# Autodesk Inventor assembly: Righter
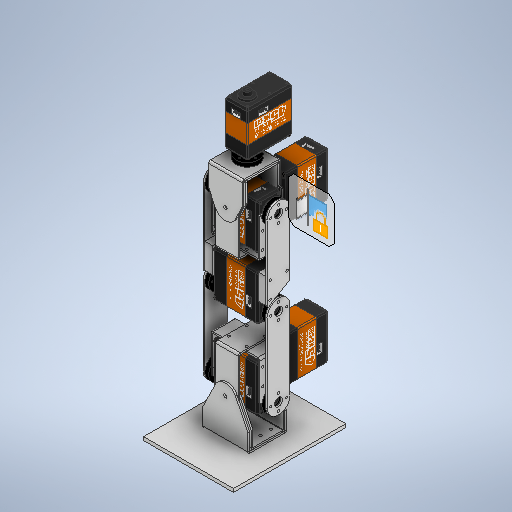
[picture p0: Inventor's stored thumbnail of the model, 512x512]
Saved by Autodesk Inventor 2025.2 (Build 292293000, 293)
## iProperties
Created: 2025-07-23
Part Number: Righter
Document SubType Name: Assembly
Designer: User
Author: User
## Documents named in this file (19)
- C:\Users\User\Documents\The Maverick's Files\College 3-3\로보인 프로젝트\RHp_Humanoid_ver1\Assembly\4_right_leg_true_final.iam
- C:\Users\User\Documents\The Maverick's Files\College 3-3\로보인 프로젝트\RHp_Humanoid_ver1\Part\HTD-45H, Horn\HTD-45H\HTD-45H.iam
- C:\Users\User\Documents\The Maverick's Files\College 3-3\로보인 프로젝트\RHp_Humanoid_ver1\Part\HTD-45H, Horn\Horn\Bottom Horn.ipt
- C:\Users\User\Documents\The Maverick's Files\College 3-3\로보인 프로젝트\RHp_Humanoid_ver1\Part\HTD-45H, Horn\Horn\Top Horn.ipt
- C:\Users\User\Documents\The Maverick's Files\College 3-3\로보인 프로젝트\RHp_Humanoid_ver1\Part\Frame\Leg\Right Leg\axis_7_top_frame.ipt
- C:\Users\User\Documents\The Maverick's Files\College 3-3\로보인 프로젝트\RHp_Humanoid_ver1\Part\Frame\Leg\Right Leg\axis_9_bottom_frame.ipt
- C:\Users\User\Documents\The Maverick's Files\College 3-3\로보인 프로젝트\RHp_Humanoid_ver1\Part\Frame\Leg\Right Leg\axis_7_supplement_frame.ipt
- C:\Users\User\Documents\The Maverick's Files\College 3-3\로보인 프로젝트\RHp_Humanoid_ver1\Part\Frame\Leg\Right Leg\axis_8_bottom_frame.ipt
- C:\Users\User\Documents\The Maverick's Files\College 3-3\로보인 프로젝트\RHp_Humanoid_ver1\Part\Frame\Leg\Right Leg\axis_8_10_connector_frame_non_powered.ipt
- C:\Users\User\Documents\The Maverick's Files\College 3-3\로보인 프로젝트\RHp_Humanoid_ver1\Part\Frame\Leg\Right Leg\axis_8_10_connector_frame_powered.ipt
- C:\Users\User\Documents\The Maverick's Files\College 3-3\로보인 프로젝트\RHp_Humanoid_ver1\Part\Frame\Leg\3D_printed_part_non_powered.ipt
- C:\Users\User\Documents\The Maverick's Files\College 3-3\로보인 프로젝트\RHp_Humanoid_ver1\Part\Frame\Leg\3D_printed_part_powered.ipt
- C:\Users\User\Documents\The Maverick's Files\College 3-3\로보인 프로젝트\RHp_Humanoid_ver1\Part\Frame\Leg\Right Leg\axis_10_11-connector_frame_non_powered.ipt
- C:\Users\User\Documents\The Maverick's Files\College 3-3\로보인 프로젝트\RHp_Humanoid_ver1\Part\Frame\Leg\Right Leg\axis_10_11-connector_frame_powered.ipt
- C:\Users\User\Documents\The Maverick's Files\College 3-3\로보인 프로젝트\RHp_Humanoid_ver1\Part\Frame\Leg\Right Leg\axis_11_top_frame.ipt
- C:\Users\User\Documents\The Maverick's Files\College 3-3\로보인 프로젝트\RHp_Humanoid_ver1\Part\Frame\Leg\Right Leg\axis_12_top_frame.ipt
- C:\Users\User\Documents\The Maverick's Files\College 3-3\로보인 프로젝트\RHp_Humanoid_ver1\Part\Frame\Leg\Right Leg\axis_12_bottom_frame(top).ipt
- C:\Users\User\Documents\The Maverick's Files\College 3-3\로보인 프로젝트\RHp_Humanoid_ver1\Part\Frame\Leg\Right Leg\axis_12_supplement_frame.ipt
- C:\Users\User\Documents\The Maverick's Files\College 3-3\로보인 프로젝트\RHp_Humanoid_ver1\Part\Frame\Leg\Right Leg\axis_12_bottom_frame(bottom).ipt
## Components (30 placed, 18 different names)
1. HTD-45H:1 [sub-assembly] — Rotational:10
2. HTD-45H:2 [sub-assembly] — Rotational:2, Rigid:5
3. HTD-45H:3 [sub-assembly] — Rigid:6, Rotational:3, Rotational:4
4. HTD-45H:4 [sub-assembly] — Rotational:5, Rotational:6, Rigid:26, Rigid:27
5. HTD-45H:5 [sub-assembly] — Rigid:16, Rotational:7, Rotational:8
6. HTD-45H:6 [sub-assembly] — Rotational:9, Rigid:19
7. Bottom Horn:3 — Rotational:3, Rigid:24
8. Bottom Horn:4 — Rotational:5, Rigid:15
9. Bottom Horn:5 — Rotational:8, Rigid:18
10. Top Horn:1 — Rigid:1, Rotational:10
11. Top Horn:2 — Rotational:2, Rigid:2
12. Top Horn:3 — Rotational:4, Rigid:9
13. Top Horn:4 — Rotational:6, Rigid:14
14. Top Horn:5 — Rotational:7, Rigid:17
15. Top Horn:6 — Rotational:9, Rigid:28
16. axis_7_top_frame:1 — Rigid:1, Rigid:2, Rigid:4
17. axis_9_bottom_frame:1 — Rigid:5, Rigid:7
18. axis_7_supplement_frame:1 — Rigid:4
19. axis_8_bottom_frame:1 — Rigid:6, Rigid:7
20. axis_8_10_connector_frame_powered:1 — Rigid:9, Rigid:11
21. axis_8_10_connector_frame_non_powered:1 — Rigid:24, Rigid:25
22. 3D_printed_part_powered:1 — Rigid:11, Rigid:26
23. 3D_printed_part_non_powered:1 — Rigid:25, Rigid:27
24. axis_10_11-connector_frame_powered:1 — Rigid:14, Rigid:17
25. axis_10_11-connector_frame_non_powered:1 — Rigid:15, Rigid:18
26. axis_11_top_frame:1 — Rigid:16, Rigid:21
27. axis_12_top_frame:1 — Rigid:19, Rigid:21
28. axis_12_bottom_frame(top):1 — Rigid:23, Rigid:28, Rigid:29
29. axis_12_supplement_frame:1 — Rigid:29
30. axis_12_bottom_frame(bottom):1 — Rigid:23
## Relationships (31: WeldJoint 22, RevoluteJoint 9)
- Rigid:1 [WeldJoint]: Top Horn:1 ↔ axis_7_top_frame:1
- Rotational:2 [RevoluteJoint]: HTD-45H:2 ↔ Top Horn:2
- Rigid:2 [WeldJoint]: Top Horn:2 ↔ axis_7_top_frame:1
- Rigid:4 [WeldJoint]: axis_7_top_frame:1 ↔ axis_7_supplement_frame:1
- Rigid:5 [WeldJoint]: HTD-45H:2 ↔ axis_9_bottom_frame:1
- Rigid:6 [WeldJoint]: HTD-45H:3 ↔ axis_8_bottom_frame:1
- Rigid:7 [WeldJoint]: axis_9_bottom_frame:1 ↔ axis_8_bottom_frame:1
- Rotational:3 [RevoluteJoint]: HTD-45H:3 ↔ Bottom Horn:3
- Rotational:4 [RevoluteJoint]: HTD-45H:3 ↔ Top Horn:3
- Rigid:9 [WeldJoint]: Top Horn:3 ↔ axis_8_10_connector_frame_powered:1
- Rigid:11 [WeldJoint]: axis_8_10_connector_frame_powered:1 ↔ 3D_printed_part_powered:1
- Rotational:5 [RevoluteJoint]: HTD-45H:4 ↔ Bottom Horn:4
- Rotational:6 [RevoluteJoint]: HTD-45H:4 ↔ Top Horn:4
- Rigid:15 [WeldJoint]: Bottom Horn:4 ↔ axis_10_11-connector_frame_non_powered:1
- Rigid:14 [WeldJoint]: Top Horn:4 ↔ axis_10_11-connector_frame_powered:1
- Rigid:16 [WeldJoint]: HTD-45H:5 ↔ axis_11_top_frame:1
- Rotational:7 [RevoluteJoint]: HTD-45H:5 ↔ Top Horn:5
- Rotational:8 [RevoluteJoint]: HTD-45H:5 ↔ Bottom Horn:5
- Rigid:17 [WeldJoint]: Top Horn:5 ↔ axis_10_11-connector_frame_powered:1
- Rigid:18 [WeldJoint]: Bottom Horn:5 ↔ axis_10_11-connector_frame_non_powered:1
- Rotational:9 [RevoluteJoint]: HTD-45H:6 ↔ Top Horn:6
- Rigid:19 [WeldJoint]: HTD-45H:6 ↔ axis_12_top_frame:1
- Rigid:21 [WeldJoint]: axis_11_top_frame:1 ↔ axis_12_top_frame:1
- Rigid:23 [WeldJoint]: axis_12_bottom_frame(top):1 ↔ axis_12_bottom_frame(bottom):1
- Rotational:10 [RevoluteJoint]: HTD-45H:1 ↔ Top Horn:1
- Rigid:24 [WeldJoint]: Bottom Horn:3 ↔ axis_8_10_connector_frame_non_powered:1
- Rigid:25 [WeldJoint]: axis_8_10_connector_frame_non_powered:1 ↔ 3D_printed_part_non_powered:1
- Rigid:26 [WeldJoint]: HTD-45H:4 ↔ 3D_printed_part_powered:1
- Rigid:27 [WeldJoint]: HTD-45H:4 ↔ 3D_printed_part_non_powered:1
- Rigid:28 [WeldJoint]: Top Horn:6 ↔ axis_12_bottom_frame(top):1
- Rigid:29 [WeldJoint]: axis_12_bottom_frame(top):1 ↔ axis_12_supplement_frame:1
